# Autodesk Inventor assembly: main
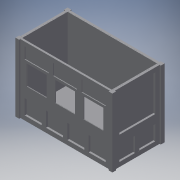
[picture p0: Inventor's stored thumbnail of the model, 180x180]
Saved by Autodesk Inventor 2017 (Build 210142000, 142)
## iProperties
Created: 2019-05-05
Part Number: main
Document SubType Name: Assembly
Designer: Roman
Author: Roman
## Documents named in this file (6)
- C:\Users\Roman\Documents\CAD\tegu rev2\main.iam
- C:\Users\Roman\Documents\CAD\tegu rev2\base\base.iam
- C:\Users\Roman\Documents\CAD\tegu rev2\floor\floor.iam
- C:\Users\Roman\Documents\CAD\tegu rev2\upper walls\long wall\upper long wall.iam
- C:\Users\Roman\Documents\CAD\tegu rev2\upper walls\short wall\short wall.iam
- C:\Users\Roman\Documents\CAD\tegu rev2\upper walls\window wall\upper window wall.iam
## Components (6 placed, 5 different names)
1. base:1 [sub-assembly] — Flush:1, Mate:1, Mate:2, Flush:3, Mate:5, Mate:6, Flush:4, Flush:5, Mate:7, Mate:8, Mate:9, Mate:10, Mate:11, Flush:7, Flush:8, Flush:9
2. floor:1 [sub-assembly] — Flush:1, Mate:1, Mate:2
3. upper long wall:2 [sub-assembly] — Flush:3, Mate:5, Mate:6
4. short wall:1 [sub-assembly] — Flush:5, Mate:7, Mate:10
5. short wall:2 [sub-assembly] — Flush:4, Mate:8, Mate:9
6. upper window wall:1 [sub-assembly] — Mate:11, Flush:7, Flush:8, Flush:9
## Relationships (16: Mate 9, Flush 7)
- Flush:1: base:1 ↔ floor:1
- Mate:1: base:1 ↔ floor:1
- Mate:2: base:1 ↔ floor:1
- Flush:3: base:1 ↔ upper long wall:2
- Mate:5: base:1 ↔ upper long wall:2
- Mate:6: base:1 ↔ upper long wall:2
- Flush:4: base:1 ↔ short wall:2
- Flush:5: base:1 ↔ short wall:1
- Mate:7: base:1 ↔ short wall:1
- Mate:8: base:1 ↔ short wall:2
- Mate:9: base:1 ↔ short wall:2
- Mate:10: base:1 ↔ short wall:1
- Mate:11: base:1 ↔ upper window wall:1
- Flush:7: base:1 ↔ upper window wall:1
- Flush:8: base:1 ↔ upper window wall:1
- Flush:9 (12.7 mm): base:1 ↔ upper window wall:1
